# Autodesk Inventor assembly: MotorClip
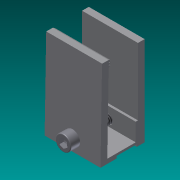
[picture p0: Inventor's stored thumbnail of the model, 180x180]
Saved by Autodesk Inventor 2013 (Build 170138000, 138)
## iProperties
Created: 2013-08-16
Part Number: MotorClip
Document SubType Name: Assembly
Designer: Sawaiz
Author: Sawaiz
## Documents named in this file (4)
- S:\Sawaiz\Documents\3D Modeling\Inventor\PolarGraph\MotorClip.iam
- S:\Sawaiz\Documents\3D Modeling\Inventor\PolarGraph\MotorClip.ipt
- S:\Sawaiz\Documents\3D Modeling\Inventor\Content Center Files\R2013\en-US\ANSI B18.3(05)\ANSI B18.3 - 8-32 UNC - 0.75(31).ipt
- S:\Sawaiz\Documents\3D Modeling\Inventor\PolarGraph\Imported Components\91841A009\91841A009.ipt
## Components (3 placed, 3 different names)
1. MotorClip:1 — Mate:1, Mate:2, Mate:3, Mate:4, Tangent:1
2. Hexagon Socket Head Cap Screw - Inch No. 8 - 32 UNC - 3/4:1 — Mate:4, Tangent:1
3. 91841A009:1 — Mate:1, Mate:2, Mate:3
## Relationships (5: Mate 4, Tangent 1)
- Mate:1: MotorClip:1 ↔ 91841A009:1
- Mate:2: MotorClip:1 ↔ 91841A009:1
- Mate:3: MotorClip:1 ↔ 91841A009:1
- Mate:4: MotorClip:1 ↔ Hexagon Socket Head Cap Screw - Inch No. 8 - 32 UNC - 3/4:1
- Tangent:1: MotorClip:1 ↔ Hexagon Socket Head Cap Screw - Inch No. 8 - 32 UNC - 3/4:1
